# Autodesk Inventor assembly: dormerScaffolding
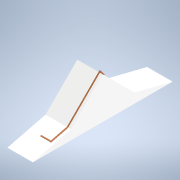
[picture p0: Inventor's stored thumbnail of the model, 180x180]
Saved by Autodesk Inventor 2021.1 (Build 251245000, 245)
## iProperties
Created: 2020-08-29
Part Number: dormerScaffolding
Document SubType Name: Assembly
Designer: robst
Author: robst
## Documents named in this file (3)
- C:\git\CAD-Development\robSteele\HouseProjects\dormerScaffolding\dormerScaffolding.iam
- C:\git\CAD-Development\robSteele\HouseProjects\dormerScaffolding\roof.ipt
- C:\git\CAD-Development\robSteele\HouseProjects\dormerScaffolding\side1.ipt
## Components (2 placed, 2 different names)
1. roof:1 — Mate:1
2. side1:1 — Mate:1
## Relationships (1: Mate 1)
- Mate:1: roof:1 ↔ side1:1
